# Autodesk Inventor assembly: SG90 - Micro Servo 9g - Tower Pro
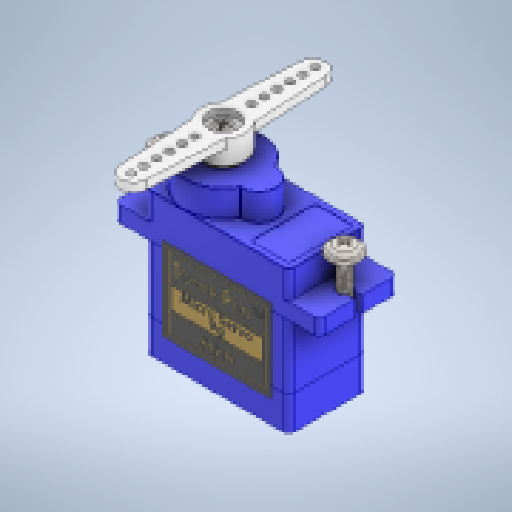
[picture p0: Inventor's stored thumbnail of the model, 512x512]
Saved by Autodesk Inventor 2026.1 (Build 301233000, 233)
## iProperties
Created: 2019-03-11
Part Number: SG90 - Micro Servo 9g - Tower Pro
Description: STEP AP214
Document SubType Name: Assembly
Designer: chris
Sending System: SolidWorks 2018
Preprocessor: SwSTEP 2.0
Title: SG90 - Micro Servo 9g - Tower Pro.STEP
Revision Number: ANY
## Documents named in this file (5)
- C:\Users\chris\Documents\Inventor\RHp_Humanoid_ver1\Part_Body\Other Parts\head\SG90 - Micro Servo 9g - Tower Pro\SG90 - Micro Servo 9g - Tower Pro\SG90 - Micro Servo 9g - Tower Pro - top.iam
- C:\Users\chris\Documents\Inventor\RHp_Humanoid_ver1\Part_Body\Other Parts\head\SG90 - Micro Servo 9g - Tower Pro\SG90 - Micro Servo 9g - Tower Pro\SG90 - Micro Servo 9g - Tower Pro.1_Pea.ipt
- C:\Users\chris\Documents\Inventor\RHp_Humanoid_ver1\Part_Body\Other Parts\head\SG90 - Micro Servo 9g - Tower Pro\SG90 - Micro Servo 9g - Tower Pro\SG90 - Micro Servo 9g - Tower Pro.3_Pea.ipt
- C:\Users\chris\Documents\Inventor\RHp_Humanoid_ver1\Part_Body\Other Parts\head\SG90 - Micro Servo 9g - Tower Pro\SG90 - Micro Servo 9g - Tower Pro\SG90 - Micro Servo 9g - Tower Pro.5_BS EN ISO 7045 - M2 x 8 - Z - 8S.ipt
- C:\Users\chris\Documents\Inventor\RHp_Humanoid_ver1\Part_Body\Other Parts\head\SG90 - Micro Servo 9g - Tower Pro\SG90 - Micro Servo 9g - Tower Pro\SG90 - Micro Servo 9g - Tower Pro.6_BS EN ISO 7045 - M2 x 4 - Z - 4S.ipt
## Components (5 placed, 5 different names)
1. SG90 - Micro Servo 9g - Tower Pro.1_Pea_1 — Rotational:1, Insert:1, Insert:2
2. SG90 - Micro Servo 9g - Tower Pro.3_Pea_3 — Rotational:1, Rigid:1
3. SG90 - Micro Servo 9g - Tower Pro.5_BS EN ISO 7045 - M2 x 8 - Z - 8S_6 — Insert:1
4. SG90 - Micro Servo 9g - Tower Pro.6_BS EN ISO 7045 - M2 x 4 - Z - 4S_7 — Rigid:1
5. SG90 - Micro Servo 9g - Tower Pro.5_BS EN ISO 7045 - M2 x 8 - Z - 8S:3 — Insert:2
## Relationships (4: Insert 2, RevoluteJoint 1, WeldJoint 1)
- Rotational:1 [RevoluteJoint]: SG90 - Micro Servo 9g - Tower Pro.1_Pea_1 ↔ SG90 - Micro Servo 9g - Tower Pro.3_Pea_3
- Rigid:1 [WeldJoint]: SG90 - Micro Servo 9g - Tower Pro.3_Pea_3 ↔ SG90 - Micro Servo 9g - Tower Pro.6_BS EN ISO 7045 - M2 x 4 - Z - 4S_7
- Insert:1 (7.4 mm): SG90 - Micro Servo 9g - Tower Pro.1_Pea_1 ↔ SG90 - Micro Servo 9g - Tower Pro.5_BS EN ISO 7045 - M2 x 8 - Z - 8S_6
- Insert:2 (4.9 mm): SG90 - Micro Servo 9g - Tower Pro.1_Pea_1 ↔ SG90 - Micro Servo 9g - Tower Pro.5_BS EN ISO 7045 - M2 x 8 - Z - 8S:3
